# Autodesk Inventor assembly: PCB
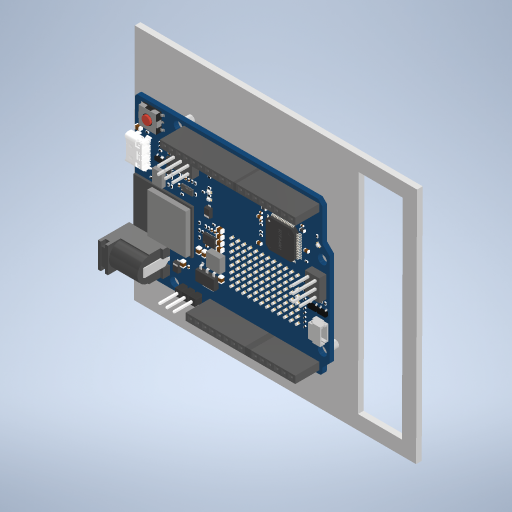
[picture p0: Inventor's stored thumbnail of the model, 512x512]
Saved by Autodesk Inventor 2024 (Build 280153020, 153B)
## iProperties
Company: Open CASCADE
Created: 2023-07-07
Part Number: PCB
Description: Open CASCADE Model
Document SubType Name: Assembly
Designer: jakub
Authority: Unknown
Sending System: Open CASCADE 7.5
Preprocessor: Open CASCADE STEP processor 7.5
Title: Open CASCADE Shape Model
Author: Author
## Documents named in this file (203)
- C:\Users\jakub\OneDrive\Pulpit\Mikołaj wydruk\UNO R4 WiFi\UNO R4 WiFi.iam
- C:\Users\jakub\OneDrive\Pulpit\Mikołaj wydruk\UNO R4 WiFi\Board.iam
- C:\Users\jakub\OneDrive\Pulpit\Mikołaj wydruk\UNO R4 WiFi\R60.iam
- C:\Users\jakub\OneDrive\Pulpit\Mikołaj wydruk\UNO R4 WiFi\R59.iam
- C:\Users\jakub\OneDrive\Pulpit\Mikołaj wydruk\UNO R4 WiFi\R20.iam
- C:\Users\jakub\OneDrive\Pulpit\Mikołaj wydruk\UNO R4 WiFi\U5.iam
- C:\Users\jakub\OneDrive\Pulpit\Mikołaj wydruk\UNO R4 WiFi\C28.iam
- C:\Users\jakub\OneDrive\Pulpit\Mikołaj wydruk\UNO R4 WiFi\R58.iam
- C:\Users\jakub\OneDrive\Pulpit\Mikołaj wydruk\UNO R4 WiFi\R57.iam
- C:\Users\jakub\OneDrive\Pulpit\Mikołaj wydruk\UNO R4 WiFi\R16.iam
- C:\Users\jakub\OneDrive\Pulpit\Mikołaj wydruk\UNO R4 WiFi\R14.iam
- C:\Users\jakub\OneDrive\Pulpit\Mikołaj wydruk\UNO R4 WiFi\R2.iam
- C:\Users\jakub\OneDrive\Pulpit\Mikołaj wydruk\UNO R4 WiFi\96.iam
- C:\Users\jakub\OneDrive\Pulpit\Mikołaj wydruk\UNO R4 WiFi\95.iam
- C:\Users\jakub\OneDrive\Pulpit\Mikołaj wydruk\UNO R4 WiFi\94.iam
- C:\Users\jakub\OneDrive\Pulpit\Mikołaj wydruk\UNO R4 WiFi\93.iam
- C:\Users\jakub\OneDrive\Pulpit\Mikołaj wydruk\UNO R4 WiFi\92.iam
- C:\Users\jakub\OneDrive\Pulpit\Mikołaj wydruk\UNO R4 WiFi\91.iam
- C:\Users\jakub\OneDrive\Pulpit\Mikołaj wydruk\UNO R4 WiFi\90.iam
- C:\Users\jakub\OneDrive\Pulpit\Mikołaj wydruk\UNO R4 WiFi\89.iam
- C:\Users\jakub\OneDrive\Pulpit\Mikołaj wydruk\UNO R4 WiFi\88.iam
- C:\Users\jakub\OneDrive\Pulpit\Mikołaj wydruk\UNO R4 WiFi\87.iam
- C:\Users\jakub\OneDrive\Pulpit\Mikołaj wydruk\UNO R4 WiFi\86.iam
- C:\Users\jakub\OneDrive\Pulpit\Mikołaj wydruk\UNO R4 WiFi\85.iam
- C:\Users\jakub\OneDrive\Pulpit\Mikołaj wydruk\UNO R4 WiFi\84.iam
- C:\Users\jakub\OneDrive\Pulpit\Mikołaj wydruk\UNO R4 WiFi\83.iam
- C:\Users\jakub\OneDrive\Pulpit\Mikołaj wydruk\UNO R4 WiFi\82.iam
- C:\Users\jakub\OneDrive\Pulpit\Mikołaj wydruk\UNO R4 WiFi\81.iam
- C:\Users\jakub\OneDrive\Pulpit\Mikołaj wydruk\UNO R4 WiFi\80.iam
- C:\Users\jakub\OneDrive\Pulpit\Mikołaj wydruk\UNO R4 WiFi\79.iam
- C:\Users\jakub\OneDrive\Pulpit\Mikołaj wydruk\UNO R4 WiFi\78.iam
- C:\Users\jakub\OneDrive\Pulpit\Mikołaj wydruk\UNO R4 WiFi\77.iam
- C:\Users\jakub\OneDrive\Pulpit\Mikołaj wydruk\UNO R4 WiFi\76.iam
- C:\Users\jakub\OneDrive\Pulpit\Mikołaj wydruk\UNO R4 WiFi\75.iam
- C:\Users\jakub\OneDrive\Pulpit\Mikołaj wydruk\UNO R4 WiFi\74.iam
- C:\Users\jakub\OneDrive\Pulpit\Mikołaj wydruk\UNO R4 WiFi\73.iam
- C:\Users\jakub\OneDrive\Pulpit\Mikołaj wydruk\UNO R4 WiFi\72.iam
- C:\Users\jakub\OneDrive\Pulpit\Mikołaj wydruk\UNO R4 WiFi\71.iam
- C:\Users\jakub\OneDrive\Pulpit\Mikołaj wydruk\UNO R4 WiFi\70.iam
- C:\Users\jakub\OneDrive\Pulpit\Mikołaj wydruk\UNO R4 WiFi\69.iam
- C:\Users\jakub\OneDrive\Pulpit\Mikołaj wydruk\UNO R4 WiFi\68.iam
- C:\Users\jakub\OneDrive\Pulpit\Mikołaj wydruk\UNO R4 WiFi\67.iam
- C:\Users\jakub\OneDrive\Pulpit\Mikołaj wydruk\UNO R4 WiFi\66.iam
- C:\Users\jakub\OneDrive\Pulpit\Mikołaj wydruk\UNO R4 WiFi\65.iam
- C:\Users\jakub\OneDrive\Pulpit\Mikołaj wydruk\UNO R4 WiFi\64.iam
- C:\Users\jakub\OneDrive\Pulpit\Mikołaj wydruk\UNO R4 WiFi\63.iam
- C:\Users\jakub\OneDrive\Pulpit\Mikołaj wydruk\UNO R4 WiFi\62.iam
- C:\Users\jakub\OneDrive\Pulpit\Mikołaj wydruk\UNO R4 WiFi\61.iam
- C:\Users\jakub\OneDrive\Pulpit\Mikołaj wydruk\UNO R4 WiFi\60.iam
- C:\Users\jakub\OneDrive\Pulpit\Mikołaj wydruk\UNO R4 WiFi\59.iam
- C:\Users\jakub\OneDrive\Pulpit\Mikołaj wydruk\UNO R4 WiFi\58.iam
- C:\Users\jakub\OneDrive\Pulpit\Mikołaj wydruk\UNO R4 WiFi\57.iam
- C:\Users\jakub\OneDrive\Pulpit\Mikołaj wydruk\UNO R4 WiFi\56.iam
- C:\Users\jakub\OneDrive\Pulpit\Mikołaj wydruk\UNO R4 WiFi\U6.iam
- C:\Users\jakub\OneDrive\Pulpit\Mikołaj wydruk\UNO R4 WiFi\U2.iam
- C:\Users\jakub\OneDrive\Pulpit\Mikołaj wydruk\UNO R4 WiFi\C30.iam
- C:\Users\jakub\OneDrive\Pulpit\Mikołaj wydruk\UNO R4 WiFi\C29.iam
- C:\Users\jakub\OneDrive\Pulpit\Mikołaj wydruk\UNO R4 WiFi\R3.iam
- C:\Users\jakub\OneDrive\Pulpit\Mikołaj wydruk\UNO R4 WiFi\M1.iam
- C:\Users\jakub\OneDrive\Pulpit\Mikołaj wydruk\UNO R4 WiFi\F1.iam
- C:\Users\jakub\OneDrive\Pulpit\Mikołaj wydruk\UNO R4 WiFi\R52.iam
- C:\Users\jakub\OneDrive\Pulpit\Mikołaj wydruk\UNO R4 WiFi\R26.iam
- C:\Users\jakub\OneDrive\Pulpit\Mikołaj wydruk\UNO R4 WiFi\R12.iam
- C:\Users\jakub\OneDrive\Pulpit\Mikołaj wydruk\UNO R4 WiFi\R11.iam
- C:\Users\jakub\OneDrive\Pulpit\Mikołaj wydruk\UNO R4 WiFi\R10.iam
- C:\Users\jakub\OneDrive\Pulpit\Mikołaj wydruk\UNO R4 WiFi\R9.iam
- C:\Users\jakub\OneDrive\Pulpit\Mikołaj wydruk\UNO R4 WiFi\Q2.iam
- C:\Users\jakub\OneDrive\Pulpit\Mikołaj wydruk\UNO R4 WiFi\Q1.iam
- C:\Users\jakub\OneDrive\Pulpit\Mikołaj wydruk\UNO R4 WiFi\J2.iam
- C:\Users\jakub\OneDrive\Pulpit\Mikołaj wydruk\UNO R4 WiFi\R13.iam
- C:\Users\jakub\OneDrive\Pulpit\Mikołaj wydruk\UNO R4 WiFi\R47.iam
- C:\Users\jakub\OneDrive\Pulpit\Mikołaj wydruk\UNO R4 WiFi\R48.iam
- C:\Users\jakub\OneDrive\Pulpit\Mikołaj wydruk\UNO R4 WiFi\R46.iam
- C:\Users\jakub\OneDrive\Pulpit\Mikołaj wydruk\UNO R4 WiFi\R45.iam
- C:\Users\jakub\OneDrive\Pulpit\Mikołaj wydruk\UNO R4 WiFi\R31.iam
- C:\Users\jakub\OneDrive\Pulpit\Mikołaj wydruk\UNO R4 WiFi\42.iam
- C:\Users\jakub\OneDrive\Pulpit\Mikołaj wydruk\UNO R4 WiFi\R34.iam
- C:\Users\jakub\OneDrive\Pulpit\Mikołaj wydruk\UNO R4 WiFi\R33.iam
- C:\Users\jakub\OneDrive\Pulpit\Mikołaj wydruk\UNO R4 WiFi\R32.iam
- C:\Users\jakub\OneDrive\Pulpit\Mikołaj wydruk\UNO R4 WiFi\R30.iam
- C:\Users\jakub\OneDrive\Pulpit\Mikołaj wydruk\UNO R4 WiFi\R29.iam
- C:\Users\jakub\OneDrive\Pulpit\Mikołaj wydruk\UNO R4 WiFi\R28.iam
- C:\Users\jakub\OneDrive\Pulpit\Mikołaj wydruk\UNO R4 WiFi\R27.iam
- C:\Users\jakub\OneDrive\Pulpit\Mikołaj wydruk\UNO R4 WiFi\54.iam
- C:\Users\jakub\OneDrive\Pulpit\Mikołaj wydruk\UNO R4 WiFi\52.iam
- C:\Users\jakub\OneDrive\Pulpit\Mikołaj wydruk\UNO R4 WiFi\50.iam
- C:\Users\jakub\OneDrive\Pulpit\Mikołaj wydruk\UNO R4 WiFi\48.iam
- C:\Users\jakub\OneDrive\Pulpit\Mikołaj wydruk\UNO R4 WiFi\46.iam
- C:\Users\jakub\OneDrive\Pulpit\Mikołaj wydruk\UNO R4 WiFi\44.iam
- C:\Users\jakub\OneDrive\Pulpit\Mikołaj wydruk\UNO R4 WiFi\55.iam
- C:\Users\jakub\OneDrive\Pulpit\Mikołaj wydruk\UNO R4 WiFi\53.iam
- C:\Users\jakub\OneDrive\Pulpit\Mikołaj wydruk\UNO R4 WiFi\51.iam
- C:\Users\jakub\OneDrive\Pulpit\Mikołaj wydruk\UNO R4 WiFi\49.iam
- C:\Users\jakub\OneDrive\Pulpit\Mikołaj wydruk\UNO R4 WiFi\47.iam
- C:\Users\jakub\OneDrive\Pulpit\Mikołaj wydruk\UNO R4 WiFi\45.iam
- C:\Users\jakub\OneDrive\Pulpit\Mikołaj wydruk\UNO R4 WiFi\43.iam
- C:\Users\jakub\OneDrive\Pulpit\Mikołaj wydruk\UNO R4 WiFi\40.iam
- C:\Users\jakub\OneDrive\Pulpit\Mikołaj wydruk\UNO R4 WiFi\38.iam
- C:\Users\jakub\OneDrive\Pulpit\Mikołaj wydruk\UNO R4 WiFi\36.iam
- C:\Users\jakub\OneDrive\Pulpit\Mikołaj wydruk\UNO R4 WiFi\34.iam
- C:\Users\jakub\OneDrive\Pulpit\Mikołaj wydruk\UNO R4 WiFi\32.iam
- C:\Users\jakub\OneDrive\Pulpit\Mikołaj wydruk\UNO R4 WiFi\41.iam
- C:\Users\jakub\OneDrive\Pulpit\Mikołaj wydruk\UNO R4 WiFi\39.iam
- C:\Users\jakub\OneDrive\Pulpit\Mikołaj wydruk\UNO R4 WiFi\37.iam
- C:\Users\jakub\OneDrive\Pulpit\Mikołaj wydruk\UNO R4 WiFi\35.iam
- C:\Users\jakub\OneDrive\Pulpit\Mikołaj wydruk\UNO R4 WiFi\33.iam
- C:\Users\jakub\OneDrive\Pulpit\Mikołaj wydruk\UNO R4 WiFi\31.iam
- C:\Users\jakub\OneDrive\Pulpit\Mikołaj wydruk\UNO R4 WiFi\30.iam
- C:\Users\jakub\OneDrive\Pulpit\Mikołaj wydruk\UNO R4 WiFi\28.iam
- C:\Users\jakub\OneDrive\Pulpit\Mikołaj wydruk\UNO R4 WiFi\26.iam
- C:\Users\jakub\OneDrive\Pulpit\Mikołaj wydruk\UNO R4 WiFi\24.iam
- C:\Users\jakub\OneDrive\Pulpit\Mikołaj wydruk\UNO R4 WiFi\22.iam
- C:\Users\jakub\OneDrive\Pulpit\Mikołaj wydruk\UNO R4 WiFi\29.iam
- C:\Users\jakub\OneDrive\Pulpit\Mikołaj wydruk\UNO R4 WiFi\27.iam
- C:\Users\jakub\OneDrive\Pulpit\Mikołaj wydruk\UNO R4 WiFi\25.iam
- C:\Users\jakub\OneDrive\Pulpit\Mikołaj wydruk\UNO R4 WiFi\23.iam
- C:\Users\jakub\OneDrive\Pulpit\Mikołaj wydruk\UNO R4 WiFi\21.iam
- C:\Users\jakub\OneDrive\Pulpit\Mikołaj wydruk\UNO R4 WiFi\20.iam
- C:\Users\jakub\OneDrive\Pulpit\Mikołaj wydruk\UNO R4 WiFi\18.iam
- C:\Users\jakub\OneDrive\Pulpit\Mikołaj wydruk\UNO R4 WiFi\16.iam
- C:\Users\jakub\OneDrive\Pulpit\Mikołaj wydruk\UNO R4 WiFi\14.iam
- C:\Users\jakub\OneDrive\Pulpit\Mikołaj wydruk\UNO R4 WiFi\19.iam
- C:\Users\jakub\OneDrive\Pulpit\Mikołaj wydruk\UNO R4 WiFi\17.iam
- C:\Users\jakub\OneDrive\Pulpit\Mikołaj wydruk\UNO R4 WiFi\15.iam
- C:\Users\jakub\OneDrive\Pulpit\Mikołaj wydruk\UNO R4 WiFi\13.iam
- C:\Users\jakub\OneDrive\Pulpit\Mikołaj wydruk\UNO R4 WiFi\12.iam
- C:\Users\jakub\OneDrive\Pulpit\Mikołaj wydruk\UNO R4 WiFi\10.iam
- C:\Users\jakub\OneDrive\Pulpit\Mikołaj wydruk\UNO R4 WiFi\8.iam
- C:\Users\jakub\OneDrive\Pulpit\Mikołaj wydruk\UNO R4 WiFi\11.iam
- C:\Users\jakub\OneDrive\Pulpit\Mikołaj wydruk\UNO R4 WiFi\9.iam
- C:\Users\jakub\OneDrive\Pulpit\Mikołaj wydruk\UNO R4 WiFi\7.iam
- C:\Users\jakub\OneDrive\Pulpit\Mikołaj wydruk\UNO R4 WiFi\6.iam
- C:\Users\jakub\OneDrive\Pulpit\Mikołaj wydruk\UNO R4 WiFi\4.iam
- C:\Users\jakub\OneDrive\Pulpit\Mikołaj wydruk\UNO R4 WiFi\5.iam
- C:\Users\jakub\OneDrive\Pulpit\Mikołaj wydruk\UNO R4 WiFi\3.iam
- C:\Users\jakub\OneDrive\Pulpit\Mikołaj wydruk\UNO R4 WiFi\2.iam
- C:\Users\jakub\OneDrive\Pulpit\Mikołaj wydruk\UNO R4 WiFi\1.iam
- C:\Users\jakub\OneDrive\Pulpit\Mikołaj wydruk\UNO R4 WiFi\R35.iam
- C:\Users\jakub\OneDrive\Pulpit\Mikołaj wydruk\UNO R4 WiFi\Q3.iam
- C:\Users\jakub\OneDrive\Pulpit\Mikołaj wydruk\UNO R4 WiFi\D1.iam
- C:\Users\jakub\OneDrive\Pulpit\Mikołaj wydruk\UNO R4 WiFi\R42.iam
- C:\Users\jakub\OneDrive\Pulpit\Mikołaj wydruk\UNO R4 WiFi\JOFF.iam
- C:\Users\jakub\OneDrive\Pulpit\Mikołaj wydruk\UNO R4 WiFi\C5.iam
- C:\Users\jakub\OneDrive\Pulpit\Mikołaj wydruk\UNO R4 WiFi\C18.iam
- C:\Users\jakub\OneDrive\Pulpit\Mikołaj wydruk\UNO R4 WiFi\C17.iam
- C:\Users\jakub\OneDrive\Pulpit\Mikołaj wydruk\UNO R4 WiFi\J6.iam
- C:\Users\jakub\OneDrive\Pulpit\Mikołaj wydruk\UNO R4 WiFi\C10.iam
- C:\Users\jakub\OneDrive\Pulpit\Mikołaj wydruk\UNO R4 WiFi\U4.iam
- C:\Users\jakub\OneDrive\Pulpit\Mikołaj wydruk\UNO R4 WiFi\C24.iam
- C:\Users\jakub\OneDrive\Pulpit\Mikołaj wydruk\UNO R4 WiFi\C25.iam
- C:\Users\jakub\OneDrive\Pulpit\Mikołaj wydruk\UNO R4 WiFi\C26.iam
- C:\Users\jakub\OneDrive\Pulpit\Mikołaj wydruk\UNO R4 WiFi\U3.iam
- C:\Users\jakub\OneDrive\Pulpit\Mikołaj wydruk\UNO R4 WiFi\U1.iam
- C:\Users\jakub\OneDrive\Pulpit\Mikołaj wydruk\UNO R4 WiFi\R23.iam
- C:\Users\jakub\OneDrive\Pulpit\Mikołaj wydruk\UNO R4 WiFi\R40.iam
- C:\Users\jakub\OneDrive\Pulpit\Mikołaj wydruk\UNO R4 WiFi\R38.iam
- C:\Users\jakub\OneDrive\Pulpit\Mikołaj wydruk\UNO R4 WiFi\R36.iam
- C:\Users\jakub\OneDrive\Pulpit\Mikołaj wydruk\UNO R4 WiFi\R44.iam
- C:\Users\jakub\OneDrive\Pulpit\Mikołaj wydruk\UNO R4 WiFi\R43.iam
- C:\Users\jakub\OneDrive\Pulpit\Mikołaj wydruk\UNO R4 WiFi\R7.iam
- C:\Users\jakub\OneDrive\Pulpit\Mikołaj wydruk\UNO R4 WiFi\R1.iam
- C:\Users\jakub\OneDrive\Pulpit\Mikołaj wydruk\UNO R4 WiFi\L3.iam
- C:\Users\jakub\OneDrive\Pulpit\Mikołaj wydruk\UNO R4 WiFi\L2.iam
- C:\Users\jakub\OneDrive\Pulpit\Mikołaj wydruk\UNO R4 WiFi\L1.iam
- C:\Users\jakub\OneDrive\Pulpit\Mikołaj wydruk\UNO R4 WiFi\C16.iam
- C:\Users\jakub\OneDrive\Pulpit\Mikołaj wydruk\UNO R4 WiFi\C11.iam
- C:\Users\jakub\OneDrive\Pulpit\Mikołaj wydruk\UNO R4 WiFi\C19.iam
- C:\Users\jakub\OneDrive\Pulpit\Mikołaj wydruk\UNO R4 WiFi\C14.iam
- C:\Users\jakub\OneDrive\Pulpit\Mikołaj wydruk\UNO R4 WiFi\C15.iam
- C:\Users\jakub\OneDrive\Pulpit\Mikołaj wydruk\UNO R4 WiFi\C13.iam
- C:\Users\jakub\OneDrive\Pulpit\Mikołaj wydruk\UNO R4 WiFi\C12.iam
- C:\Users\jakub\OneDrive\Pulpit\Mikołaj wydruk\UNO R4 WiFi\C20.iam
- C:\Users\jakub\OneDrive\Pulpit\Mikołaj wydruk\UNO R4 WiFi\C9.iam
- C:\Users\jakub\OneDrive\Pulpit\Mikołaj wydruk\UNO R4 WiFi\C8.iam
- C:\Users\jakub\OneDrive\Pulpit\Mikołaj wydruk\UNO R4 WiFi\C6.iam
- C:\Users\jakub\OneDrive\Pulpit\Mikołaj wydruk\UNO R4 WiFi\C3.iam
- C:\Users\jakub\OneDrive\Pulpit\Mikołaj wydruk\UNO R4 WiFi\C2.iam
- C:\Users\jakub\OneDrive\Pulpit\Mikołaj wydruk\UNO R4 WiFi\R51.iam
- C:\Users\jakub\OneDrive\Pulpit\Mikołaj wydruk\UNO R4 WiFi\R50.iam
- C:\Users\jakub\OneDrive\Pulpit\Mikołaj wydruk\UNO R4 WiFi\R15.iam
- C:\Users\jakub\OneDrive\Pulpit\Mikołaj wydruk\UNO R4 WiFi\R18.iam
- C:\Users\jakub\OneDrive\Pulpit\Mikołaj wydruk\UNO R4 WiFi\R24.iam
- C:\Users\jakub\OneDrive\Pulpit\Mikołaj wydruk\UNO R4 WiFi\R19.iam
- C:\Users\jakub\OneDrive\Pulpit\Mikołaj wydruk\UNO R4 WiFi\R49.iam
- C:\Users\jakub\OneDrive\Pulpit\Mikołaj wydruk\UNO R4 WiFi\R25.iam
- C:\Users\jakub\OneDrive\Pulpit\Mikołaj wydruk\UNO R4 WiFi\DL3.iam
- C:\Users\jakub\OneDrive\Pulpit\Mikołaj wydruk\UNO R4 WiFi\C21.iam
- C:\Users\jakub\OneDrive\Pulpit\Mikołaj wydruk\UNO R4 WiFi\R22.iam
- C:\Users\jakub\OneDrive\Pulpit\Mikołaj wydruk\UNO R4 WiFi\DL2.iam
- C:\Users\jakub\OneDrive\Pulpit\Mikołaj wydruk\UNO R4 WiFi\DL1.iam
- C:\Users\jakub\OneDrive\Pulpit\Mikołaj wydruk\UNO R4 WiFi\DL4.iam
- C:\Users\jakub\OneDrive\Pulpit\Mikołaj wydruk\UNO R4 WiFi\R17.iam
- C:\Users\jakub\OneDrive\Pulpit\Mikołaj wydruk\UNO R4 WiFi\C7.iam
- C:\Users\jakub\OneDrive\Pulpit\Mikołaj wydruk\UNO R4 WiFi\J5.iam
- C:\Users\jakub\OneDrive\Pulpit\Mikołaj wydruk\UNO R4 WiFi\D2.iam
- C:\Users\jakub\OneDrive\Pulpit\Mikołaj wydruk\UNO R4 WiFi\D3.iam
- C:\Users\jakub\OneDrive\Pulpit\Mikołaj wydruk\UNO R4 WiFi\J3.iam
- C:\Users\jakub\OneDrive\Pulpit\Mikołaj wydruk\UNO R4 WiFi\PB1.iam
- C:\Users\jakub\OneDrive\Pulpit\Mikołaj wydruk\UNO R4 WiFi\R39.iam
- C:\Users\jakub\OneDrive\Pulpit\Mikołaj wydruk\UNO R4 WiFi\J1.iam
- C:\Users\jakub\OneDrive\Pulpit\Mikołaj wydruk\UNO R4 WiFi\JDIGITAL.iam
- C:\Users\jakub\OneDrive\Pulpit\Mikołaj wydruk\UNO R4 WiFi\JANALOG.iam
- C:\Users\jakub\OneDrive\Pulpit\Mikołaj wydruk\gora.ipt
## Components (202 placed, 202 different names)
1. Board_992 [sub-assembly] — Obrotowe:1
2. R60_994 [sub-assembly]
3. R59_996 [sub-assembly]
4. R20_998 [sub-assembly]
5. U5_1006 [sub-assembly]
6. C28_1008 [sub-assembly]
7. R58_1010 [sub-assembly]
8. R57_1012 [sub-assembly]
9. R16_1014 [sub-assembly]
10. R14_1016 [sub-assembly]
11. R2_1018 [sub-assembly]
12. 96_1020 [sub-assembly]
13. 95_1022 [sub-assembly]
14. 94_1024 [sub-assembly]
15. 93_1026 [sub-assembly]
16. 92_1028 [sub-assembly]
17. 91_1030 [sub-assembly]
18. 90_1032 [sub-assembly]
19. 89_1034 [sub-assembly]
20. 88_1036 [sub-assembly]
21. 87_1038 [sub-assembly]
22. 86_1040 [sub-assembly]
23. 85_1042 [sub-assembly]
24. 84_1044 [sub-assembly]
25. 83_1046 [sub-assembly]
26. 82_1048 [sub-assembly]
27. 81_1050 [sub-assembly]
28. 80_1052 [sub-assembly]
29. 79_1054 [sub-assembly]
30. 78_1056 [sub-assembly]
31. 77_1058 [sub-assembly]
32. 76_1060 [sub-assembly]
33. 75_1062 [sub-assembly]
34. 74_1064 [sub-assembly]
35. 73_1066 [sub-assembly]
36. 72_1068 [sub-assembly]
37. 71_1070 [sub-assembly]
38. 70_1072 [sub-assembly]
39. 69_1074 [sub-assembly]
40. 68_1076 [sub-assembly]
41. 67_1078 [sub-assembly]
42. 66_1080 [sub-assembly]
43. 65_1082 [sub-assembly]
44. 64_1084 [sub-assembly]
45. 63_1086 [sub-assembly]
46. 62_1088 [sub-assembly]
47. 61_1090 [sub-assembly]
48. 60_1092 [sub-assembly]
49. 59_1094 [sub-assembly]
50. 58_1096 [sub-assembly]
51. 57_1098 [sub-assembly]
52. 56_1100 [sub-assembly]
53. U6_1111 [sub-assembly]
54. U2_1113 [sub-assembly]
55. C30_1115 [sub-assembly]
56. C29_1117 [sub-assembly]
57. R3_1119 [sub-assembly]
58. M1_1124 [sub-assembly]
59. F1_1127 [sub-assembly]
60. R52_1129 [sub-assembly]
61. R26_1131 [sub-assembly]
62. R12_1133 [sub-assembly]
63. R11_1135 [sub-assembly]
64. R10_1137 [sub-assembly]
65. R9_1139 [sub-assembly]
66. Q2_1141 [sub-assembly]
67. Q1_1143 [sub-assembly]
68. J2_1145 [sub-assembly]
69. R13_1147 [sub-assembly]
70. R47_1149 [sub-assembly]
71. R48_1151 [sub-assembly]
72. R46_1153 [sub-assembly]
73. R45_1155 [sub-assembly]
74. R31_1157 [sub-assembly]
75. 42_1159 [sub-assembly]
76. R34_1161 [sub-assembly]
77. R33_1163 [sub-assembly]
78. R32_1165 [sub-assembly]
79. R30_1167 [sub-assembly]
80. R29_1169 [sub-assembly]
81. R28_1171 [sub-assembly]
82. R27_1173 [sub-assembly]
83. 54_1175 [sub-assembly]
84. 52_1177 [sub-assembly]
85. 50_1179 [sub-assembly]
86. 48_1181 [sub-assembly]
87. 46_1183 [sub-assembly]
88. 44_1185 [sub-assembly]
89. 55_1187 [sub-assembly]
90. 53_1189 [sub-assembly]
91. 51_1191 [sub-assembly]
92. 49_1193 [sub-assembly]
93. 47_1195 [sub-assembly]
94. 45_1197 [sub-assembly]
95. 43_1199 [sub-assembly]
96. 40_1201 [sub-assembly]
97. 38_1203 [sub-assembly]
98. 36_1205 [sub-assembly]
99. 34_1207 [sub-assembly]
100. 32_1209 [sub-assembly]
101. 41_1211 [sub-assembly]
102. 39_1213 [sub-assembly]
103. 37_1215 [sub-assembly]
104. 35_1217 [sub-assembly]
105. 33_1219 [sub-assembly]
106. 31_1221 [sub-assembly]
107. 30_1223 [sub-assembly]
108. 28_1225 [sub-assembly]
109. 26_1227 [sub-assembly]
110. 24_1229 [sub-assembly]
111. 22_1231 [sub-assembly]
112. 29_1233 [sub-assembly]
113. 27_1235 [sub-assembly]
114. 25_1237 [sub-assembly]
115. 23_1239 [sub-assembly]
116. 21_1241 [sub-assembly]
117. 20_1243 [sub-assembly]
118. 18_1245 [sub-assembly]
119. 16_1247 [sub-assembly]
120. 14_1249 [sub-assembly]
121. 19_1251 [sub-assembly]
122. 17_1253 [sub-assembly]
123. 15_1255 [sub-assembly]
124. 13_1257 [sub-assembly]
125. 12_1259 [sub-assembly]
126. 10_1261 [sub-assembly]
127. 8_1263 [sub-assembly]
128. 11_1265 [sub-assembly]
129. 9_1267 [sub-assembly]
130. 7_1269 [sub-assembly]
131. 6_1271 [sub-assembly]
132. 4_1273 [sub-assembly]
133. 5_1275 [sub-assembly]
134. 3_1277 [sub-assembly]
135. 2_1279 [sub-assembly]
136. 1_1281 [sub-assembly]
137. R35_1283 [sub-assembly]
138. Q3_1285 [sub-assembly]
139. D1_1292 [sub-assembly]
140. R42_1294 [sub-assembly]
141. JOFF_1298 [sub-assembly]
142. C5_1300 [sub-assembly]
143. C18_1302 [sub-assembly]
144. C17_1304 [sub-assembly]
145. J6_1306 [sub-assembly]
146. C10_1308 [sub-assembly]
147. U4_1331 [sub-assembly]
148. C24_1333 [sub-assembly]
149. C25_1335 [sub-assembly]
150. C26_1337 [sub-assembly]
151. U3_1356 [sub-assembly]
152. U1_1430 [sub-assembly]
153. R23_1432 [sub-assembly]
154. R40_1434 [sub-assembly]
155. R38_1436 [sub-assembly]
156. R36_1438 [sub-assembly]
157. R44_1440 [sub-assembly]
158. R43_1442 [sub-assembly]
159. R7_1444 [sub-assembly]
160. R1_1446 [sub-assembly]
161. L3_1449 [sub-assembly]
162. L2_1451 [sub-assembly]
163. L1_1453 [sub-assembly]
164. C16_1455 [sub-assembly]
165. C11_1457 [sub-assembly]
166. C19_1459 [sub-assembly]
167. C14_1461 [sub-assembly]
168. C15_1463 [sub-assembly]
169. C13_1465 [sub-assembly]
170. C12_1467 [sub-assembly]
171. C20_1469 [sub-assembly]
172. C9_1471 [sub-assembly]
173. C8_1473 [sub-assembly]
174. C6_1475 [sub-assembly]
175. C3_1477 [sub-assembly]
176. C2_1479 [sub-assembly]
177. R51_1481 [sub-assembly]
178. R50_1483 [sub-assembly]
179. R15_1485 [sub-assembly]
180. R18_1487 [sub-assembly]
181. R24_1489 [sub-assembly]
182. R19_1491 [sub-assembly]
183. R49_1493 [sub-assembly]
184. R25_1495 [sub-assembly]
185. DL3_1497 [sub-assembly]
186. C21_1499 [sub-assembly]
187. R22_1501 [sub-assembly]
188. DL2_1503 [sub-assembly]
189. DL1_1505 [sub-assembly]
190. DL4_1507 [sub-assembly]
191. R17_1509 [sub-assembly]
192. C7_1511 [sub-assembly]
193. J5_1513 [sub-assembly]
194. D2_1515 [sub-assembly]
195. D3_1517 [sub-assembly]
196. J3_1519 [sub-assembly]
197. PB1_1521 [sub-assembly]
198. R39_1523 [sub-assembly]
199. J1_1526 [sub-assembly]
200. JDIGITAL_1531 [sub-assembly]
201. JANALOG_1536 [sub-assembly]
202. gora:1 — Obrotowe:1
## Relationships (1: RevoluteJoint 1)
- Obrotowe:1 [RevoluteJoint]: Board_992 ↔ gora:1
